# Autodesk Inventor assembly: Shooter Oct10
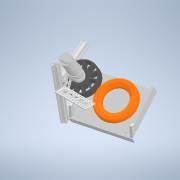
[picture p0: Inventor's stored thumbnail of the model, 180x180]
Saved by Autodesk Inventor 2020.3 (Build 243373010, 373A)
## iProperties
Created: 2020-10-10
Part Number: Shooter Oct10
Document SubType Name: Assembly
Designer: Owner
Author: Owner
## Documents named in this file (11)
- C:\Users\Owner\Documents\GitHub\CAD-2021-Ultimate_Goal\Shooter\Shooter Oct10.iam
- C:\Users\Owner\Documents\GitHub\CAD-2021-Ultimate_Goal\ServoCity\7in-Xrail.ipt
- C:\Users\Owner\Documents\GitHub\CAD-2021-Ultimate_Goal\ServoCity\555176 assembly.ipt
- C:\Users\Owner\Documents\GitHub\CAD-2021-Ultimate_Goal\ServoCity\585720.ipt
- C:\Users\Owner\Documents\GitHub\CAD-2021-Ultimate_Goal\GoBilda\5202-0002-0003 part.ipt
- C:\Users\Owner\Documents\GitHub\CAD-2021-Ultimate_Goal\Shooter\Shooter plate but for an xrail.ipt
- C:\Users\Owner\Documents\GitHub\CAD-2021-Ultimate_Goal\AndyMark\am-3563 4IN 8mm Round Compliant Wheel REV2.ipt
- C:\Users\Owner\Documents\GitHub\CAD-2021-Ultimate_Goal\ServoCity\545456.ipt
- C:\Users\Owner\Documents\GitHub\CAD-2021-Ultimate_Goal\ServoCity\545636 assembly.ipt
- C:\Users\Owner\Documents\GitHub\CAD-2021-Ultimate_Goal\AndyMark\am-4300 Ring.ipt
- C:\Users\Owner\Documents\GitHub\CAD-2021-Ultimate_Goal\ServoCity\585722.ipt
## Components (13 placed, 10 different names)
1. 7in-Xrail:1 — Mate:29
2. 585720:1 — Mate:6, Mate:7, Mate:8, Mate:26, Mate:28
3. 7in-Xrail:2 — Mate:10, Mate:11
4. 5202-0002-0003 part:1 — Mate:9, Mate:14, Mate:15, Mate:21, Mate:27
5. 555176 assembly:1 — Mate:6, Mate:7, Mate:8, Mate:9, Mate:21
6. Shooter plate but for an xrail:1 — Mate:10, Mate:11, Mate:24
7. am-3563 4IN 8mm Round Compliant Wheel REV2:1 — Mate:22, Mate:23
8. 545456:1 — Mate:13, Mate:16, Mate:17, Mate:22, Mate:23
9. 545636 assembly:1 — Mate:13, Mate:14, Mate:15, Mate:16, Mate:17
10. am-4300 Ring:1 — Mate:24
11. 7in-Xrail:3 — Mate:28, Mate:29
12. 555176 assembly:2 — Mate:26, Mate:27
13. 585722:1
## Relationships (19: Mate 19)
- Mate:6: 585720:1 ↔ 555176 assembly:1
- Mate:7: 585720:1 ↔ 555176 assembly:1
- Mate:8: 585720:1 ↔ 555176 assembly:1
- Mate:9: 5202-0002-0003 part:1 ↔ 555176 assembly:1
- Mate:10: 7in-Xrail:2 ↔ Shooter plate but for an xrail:1
- Mate:11: 7in-Xrail:2 ↔ Shooter plate but for an xrail:1
- Mate:13: 545456:1 ↔ 545636 assembly:1
- Mate:14: 5202-0002-0003 part:1 ↔ 545636 assembly:1
- Mate:15: 5202-0002-0003 part:1 ↔ 545636 assembly:1
- Mate:16: 545456:1 ↔ 545636 assembly:1
- Mate:17: 545456:1 ↔ 545636 assembly:1
- Mate:21: 5202-0002-0003 part:1 ↔ 555176 assembly:1
- Mate:22: am-3563 4IN 8mm Round Compliant Wheel REV2:1 ↔ 545456:1
- Mate:23: am-3563 4IN 8mm Round Compliant Wheel REV2:1 ↔ 545456:1
- Mate:24: Shooter plate but for an xrail:1 ↔ am-4300 Ring:1
- Mate:26: 585720:1 ↔ 555176 assembly:2
- Mate:27: 5202-0002-0003 part:1 ↔ 555176 assembly:2
- Mate:28: 585720:1 ↔ 7in-Xrail:3
- Mate:29: 7in-Xrail:1 ↔ 7in-Xrail:3
